# Autodesk Inventor assembly: Blade Assembly
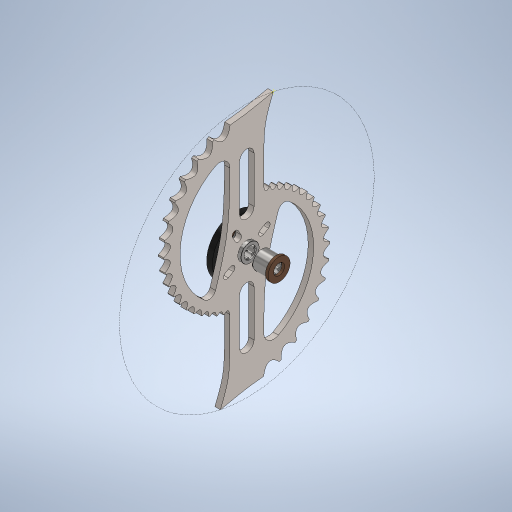
[picture p0: Inventor's stored thumbnail of the model, 512x512]
Saved by Autodesk Inventor 2023.1 (Build 271208000, 208)
## iProperties
Created: 2022-08-25
Part Number: Blade Assembly
Document SubType Name: Assembly
Designer: Nathan Cai
Mass: 59.239 g
Surface Area: 128.523 cm^2
Volume: 11.9406 cm^3
Density: 4.96116 g/cm^3
Author: Nathan Cai
## Documents named in this file (5)
- E:\Documents\Inventor\3rd Lawelle - V0.1\Blade Assembly.iam
- E:\Documents\Inventor\3rd Lawelle - V0.1\5.5in Spinner Bar R1.ipt
- E:\Documents\Inventor\3rd Lawelle - V0.1\(NRB 10mmOD 6mmID) 5905K351_Needle-Roller Bearing.ipt
- E:\Documents\Inventor\3rd Lawelle - V0.1\2011N111_Oil-Embedded Thrust Bronze Bearing.ipt
- E:\Documents\Inventor\3rd Lawelle - V0.1\Spacer.ipt
## Components (6 placed, 4 different names)
1. 5.5in Spinner Bar R1:1 — Mate:1, Flush:1, Mate:9, Mate:10
2. (NRB 10mmOD 6mmID) 5905K351_Needle-Roller Bearing:1 — Mate:1, Flush:1, Mate:2, Mate:3, Mate:6, Mate:8
3. (NRB 10mmOD 6mmID) 5905K351_Needle-Roller Bearing:2 — Mate:2, Mate:4, Mate:5
4. 2011N111_Oil-Embedded Thrust Bronze Bearing:1 — Mate:3, Mate:6, Mate:7
5. 2011N111_Oil-Embedded Thrust Bronze Bearing:2 — Mate:4, Mate:5, Mate:7
6. Spacer:1 — Mate:8, Mate:9, Mate:10
## Relationships (11: Mate 10, Flush 1)
- Mate:1: 5.5in Spinner Bar R1:1 ↔ (NRB 10mmOD 6mmID) 5905K351_Needle-Roller Bearing:1
- Flush:1 (-3.175 mm): 5.5in Spinner Bar R1:1 ↔ (NRB 10mmOD 6mmID) 5905K351_Needle-Roller Bearing:1
- Mate:2: (NRB 10mmOD 6mmID) 5905K351_Needle-Roller Bearing:1 ↔ (NRB 10mmOD 6mmID) 5905K351_Needle-Roller Bearing:2
- Mate:3: (NRB 10mmOD 6mmID) 5905K351_Needle-Roller Bearing:1 ↔ 2011N111_Oil-Embedded Thrust Bronze Bearing:1
- Mate:4: (NRB 10mmOD 6mmID) 5905K351_Needle-Roller Bearing:2 ↔ 2011N111_Oil-Embedded Thrust Bronze Bearing:2
- Mate:5: (NRB 10mmOD 6mmID) 5905K351_Needle-Roller Bearing:2 ↔ 2011N111_Oil-Embedded Thrust Bronze Bearing:2
- Mate:6: (NRB 10mmOD 6mmID) 5905K351_Needle-Roller Bearing:1 ↔ 2011N111_Oil-Embedded Thrust Bronze Bearing:1
- Mate:7 (-25.4 mm): 2011N111_Oil-Embedded Thrust Bronze Bearing:1 ↔ 2011N111_Oil-Embedded Thrust Bronze Bearing:2
- Mate:8: (NRB 10mmOD 6mmID) 5905K351_Needle-Roller Bearing:1 ↔ Spacer:1
- Mate:9: 5.5in Spinner Bar R1:1 ↔ Spacer:1
- Mate:10: 5.5in Spinner Bar R1:1 ↔ Spacer:1
